# Autodesk Inventor assembly: HW2_1_task
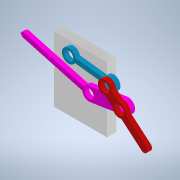
[picture p0: Inventor's stored thumbnail of the model, 180x180]
Saved by Autodesk Inventor 2022 (Build 260153000, 153)
## iProperties
Created: 2022-03-07
Part Number: HW2_1_task
Document SubType Name: Assembly
Designer: Administrator
Title: HW2_1_task v1
Author: Administrator
## Documents named in this file (5)
- C:\Users\br4ch\M-and-Ms\HW5\ANSYS\HW2_1_task.iam
- C:\Users\br4ch\M-and-Ms\HW5\ANSYS\C1.ipt
- C:\Users\br4ch\M-and-Ms\HW5\ANSYS\C2.ipt
- C:\Users\br4ch\M-and-Ms\HW5\ANSYS\C3.ipt
- C:\Users\br4ch\M-and-Ms\HW5\ANSYS\Base.ipt
## Components (4 placed, 4 different names)
1. C1:1 — Rotational:1, Rotational:2
2. C2:1 — Rotational:2, Rotational:3
3. C3:1 — Rotational:3, Rotational:4
4. Base:1 — Rotational:1, Rotational:4
## Relationships (4: RevoluteJoint 4)
- Rotational:1 [RevoluteJoint]: C1:1 ↔ Base:1
- Rotational:2 [RevoluteJoint]: C1:1 ↔ C2:1
- Rotational:3 [RevoluteJoint]: C2:1 ↔ C3:1
- Rotational:4 [RevoluteJoint]: C3:1 ↔ Base:1
